# Autodesk Inventor assembly: Assembly1
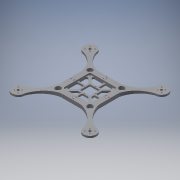
[picture p0: Inventor's stored thumbnail of the model, 180x180]
Saved by Autodesk Inventor 2016 (Build 200138000, 138)
## iProperties
Created: 2016-01-29
Part Number: Assembly1
Document SubType Name: Assembly
Designer: cemer
Author: cemer
## Documents named in this file (2)
- C:\Users\cemer\Desktop\Assembly1.iam
- C:\Users\cemer\Documents\Inventor\Drone\dron1.ipt
## Components (4 placed, 1 different names)
1. dron1:1 — Mate:1, Mate:6
2. dron1:2 — Mate:1, Mate:2, Mate:3
3. dron1:3 — Mate:2, Mate:3, Mate:4, Mate:5
4. dron1:4 — Mate:4, Mate:5, Mate:6
## Relationships (6: Mate 6)
- Mate:1: dron1:1 ↔ dron1:2
- Mate:2: dron1:2 ↔ dron1:3
- Mate:3: dron1:2 ↔ dron1:3
- Mate:4: dron1:3 ↔ dron1:4
- Mate:5: dron1:3 ↔ dron1:4
- Mate:6: dron1:1 ↔ dron1:4
